# Autodesk Inventor assembly: REVE_02-1_ASSEMBLY_RIB_CDEF_ASM
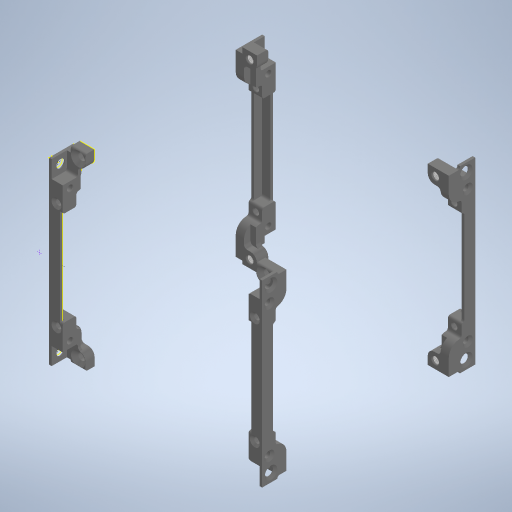
[picture p0: Inventor's stored thumbnail of the model, 512x512]
Saved by Autodesk Inventor 2023 (Build 270158000, 158)
## iProperties
Created: 2011-03-02
Part Number: REVE_02-1_ASSEMBLY_RIB_CDEF_ASM
Description: NOT SPECIFIED
Document SubType Name: Assembly
Designer: maylo
Author: maylo
Revision Number: LAST_VERSION
## Documents named in this file (6)
- E:\Dropbox\AMSAT\Cube Sat Frame Info\ISIS\REVE_02-1_ASSEMBLY_RIB_CDEF_ASM.iam
- E:\Dropbox\AMSAT\Cube Sat Frame Info\ISIS\HELICOIL_M3_1_5D.ipt
- E:\Dropbox\AMSAT\Cube Sat Frame Info\ISIS\REVD_02-1_RIB_D.ipt
- E:\Dropbox\AMSAT\Cube Sat Frame Info\ISIS\REVE_02-1_RIB_E.ipt
- E:\Dropbox\AMSAT\Cube Sat Frame Info\ISIS\REVE_02-1_RIB_C.ipt
- E:\Dropbox\AMSAT\Cube Sat Frame Info\ISIS\REVD_02-1_RIB_F.ipt
## Components (8 placed, 8 different names)
1. HELICOIL_M3_1_5D_24
2. HELICOIL_M3_1_5D_25
3. REVD_02-1_RIB_D_26 — Symmetry:1, Symmetry:2
4. REVE_02-1_RIB_E_27
5. REVE_02-1_RIB_C_28
6. HELICOIL_M3_1_5D_29
7. HELICOIL_M3_1_5D_30
8. REVD_02-1_RIB_F_31 — Symmetry:1, Symmetry:2
## Relationships (2: Symmetry 2)
- Symmetry:1: REVD_02-1_RIB_D_26 ↔ REVD_02-1_RIB_F_31
- Symmetry:2: REVD_02-1_RIB_D_26 ↔ REVD_02-1_RIB_F_31
